# Autodesk Inventor assembly: гроб для задницы цел
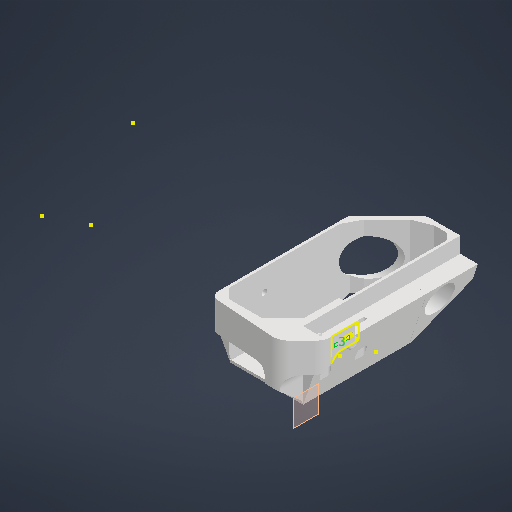
[picture p0: Inventor's stored thumbnail of the model, 512x512]
Saved by Autodesk Inventor 2025 (Build 290162000, 162)
## iProperties
Created: 2024-08-15
Part Number: гроб для задницы цел
Document SubType Name: Assembly
Designer: GameHD
Author: GameHD
## Documents named in this file (3)
- C:\Users\GameHD\Desktop\робототехника\гроб для задницы цел.iam
- C:\Users\GameHD\Desktop\робототехника\гроб для задницы.ipt
- C:\Users\GameHD\Desktop\робототехника\гроб для задницы 2 ч.ipt
## Components (2 placed, 2 different names)
1. гроб для задницы:1 — Жесткий:1
2. гроб для задницы 2 ч:1 — Жесткий:1
## Relationships (1: WeldJoint 1)
- Жесткий:1 [WeldJoint]: гроб для задницы:1 ↔ гроб для задницы 2 ч:1
